# Autodesk Inventor assembly: Collumn
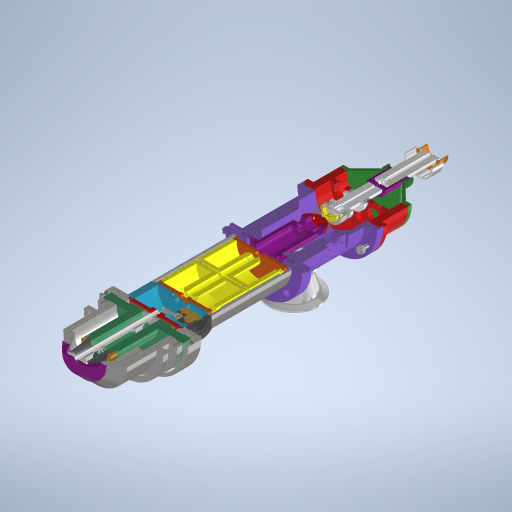
[picture p0: Inventor's stored thumbnail of the model, 512x512]
Saved by Autodesk Inventor 2023 (Build 270158000, 158)
## iProperties
Created: 2022-03-30
Part Number: Collumn
Document SubType Name: Assembly
Designer: Vinicius Miguel
Mass: 12312.5 g
Surface Area: 6705.51 cm^2
Volume: 2061.09 cm^3
Density: 5.97381 g/cm^3
Author: Vinicius Miguel
## Documents named in this file (8)
- P:\SEM-Mechanical\Collumn.iam
- P:\SEM-Mechanical\Objective.iam
- P:\SEM-Mechanical\Condensers.iam
- P:\SEM-Mechanical\008.ipt
- P:\SEM-Mechanical\Anode.iam
- P:\SEM-Mechanical\ElectronGun.iam
- P:\SEM-Mechanical\ApertureActuator.iam
- P:\SEM-Mechanical\025.ipt
## Components (7 placed, 7 different names)
1. Objective:1 [sub-assembly] — Mate:1, Flush:1, Flush:2, Mate:4, Mate:10
2. 008:1 — Mate:3, Mate:4, Mate:5, Mate:6, Rotational:2, Angle:1, Mate:17, Mate:18
3. 025:1 — Mate:17, Mate:18
4. Condensers:1 [sub-assembly] — Mate:2, Mate:5, Mate:9
5. Anode:1 [sub-assembly] — Mate:7, Mate:9, Mate:10, Mate:16, Mate:19, Mate:20
6. ElectronGun:1 [sub-assembly] — Mate:16, Mate:19, Mate:20
7. ApertureActuator:1 [sub-assembly] — Rotational:2, Angle:1
## Relationships (18: Mate 14, Flush 2, RevoluteJoint 1, Angle 1)
- Mate:1: Objective:1
- Flush:1: Objective:1
- Flush:2: Objective:1
- Mate:2: Condensers:1
- Mate:3: 008:1
- Mate:4: Objective:1 ↔ 008:1
- Mate:5: 008:1 ↔ Condensers:1
- Mate:6: 008:1
- Mate:7: Anode:1
- Mate:9: Condensers:1 ↔ Anode:1
- Mate:10: Objective:1 ↔ Anode:1
- Mate:16: Anode:1 ↔ ElectronGun:1
- Rotational:2 [RevoluteJoint]: 008:1 ↔ ApertureActuator:1
- Angle:1 (0 deg): 008:1 ↔ ApertureActuator:1
- Mate:17: 008:1 ↔ 025:1
- Mate:18: 008:1 ↔ 025:1
- Mate:19: Anode:1 ↔ ElectronGun:1
- Mate:20: Anode:1 ↔ ElectronGun:1
